# Autodesk Inventor assembly: ShakerAssembly
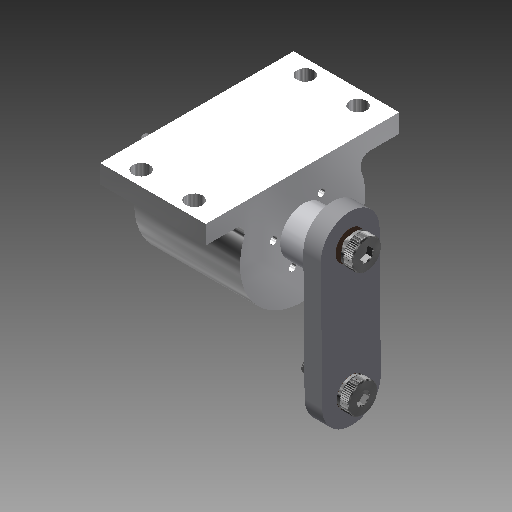
[picture p0: Inventor's stored thumbnail of the model, 512x512]
Saved by Autodesk Inventor 2017 (Build 210142000, 142)
## iProperties
Created: 2017-02-08
Part Number: ShakerAssembly
Document SubType Name: Assembly
Designer: Joseph
Author: Joseph
## Documents named in this file (8)
- C:\Users\qupec\Desktop\UMD Near Space\RockSat\ShakerCAD\ShakerAssembly.iam
- C:\Users\qupec\Desktop\UMD Near Space\RockSat\ShakerCAD\MotorMount.ipt
- C:\Users\qupec\Desktop\UMD Near Space\RockSat\ShakerCAD\Motor.ipt
- C:\Users\qupec\Desktop\UMD Near Space\RockSat\ShakerCAD\MotorArm.ipt
- C:\Users\qupec\Desktop\UMD Near Space\RockSat\ShakerCAD\RotationArm.ipt
- C:\Users\qupec\Desktop\UMD Near Space\RockSat\ShakerCAD\Bearing.ipt
- C:\Users\qupec\Desktop\UMD Near Space\RockSat\ShakerCAD\Linkage.ipt
- C:\Users\qupec\Desktop\UMD Near Space\RockSat\Motor Holder.ipt
## Components (9 placed, 7 different names)
1. MotorMount:1 — Insert:1, Insert:2, Mate:1
2. Motor:1 — Insert:1, Insert:2, Rotational:1, Mate:2, Mate:3, Mate:4, Mate:5
3. MotorArm:1 — Rotational:1, Rotational:2
4. RotationArm:1 — Rotational:2, Rotational:3
5. Bearing:1 — Rigid:1, Rotational:3
6. Bearing:2 — Rigid:2, Mate:1, Rotational:4
7. Linkage:1 — Rigid:1, Rigid:2
8. RotationArm:2 — Rotational:4
9. Motor Holder:1 — Mate:2, Mate:3, Mate:4, Mate:5
## Relationships (13: Mate 5, RevoluteJoint 4, Insert 2, WeldJoint 2)
- Insert:1: MotorMount:1 ↔ Motor:1
- Insert:2: MotorMount:1 ↔ Motor:1
- Rotational:1 [RevoluteJoint]: Motor:1 ↔ MotorArm:1
- Rotational:2 [RevoluteJoint]: MotorArm:1 ↔ RotationArm:1
- Rigid:1 [WeldJoint]: Bearing:1 ↔ Linkage:1
- Rigid:2 [WeldJoint]: Bearing:2 ↔ Linkage:1
- Rotational:3 [RevoluteJoint]: RotationArm:1 ↔ Bearing:1
- Mate:1 (-12.7 mm): MotorMount:1 ↔ Bearing:2
- Rotational:4 [RevoluteJoint]: Bearing:2 ↔ RotationArm:2
- Mate:2: Motor:1 ↔ Motor Holder:1
- Mate:3: Motor:1 ↔ Motor Holder:1
- Mate:4: Motor:1 ↔ Motor Holder:1
- Mate:5: Motor:1 ↔ Motor Holder:1
